# Autodesk Inventor assembly: segment1
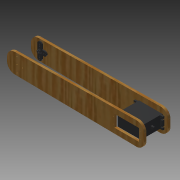
[picture p0: Inventor's stored thumbnail of the model, 180x180]
Saved by Autodesk Inventor 2013 (Build 170138000, 138)
## iProperties
Created: 2014-10-10
Part Number: segment1
Document SubType Name: Assembly
Designer: Masta
Author: Masta
## Documents named in this file (4)
- D:\DrOctopus\3D model\segment1.iam
- D:\DrOctopus\3D model\segment1a.ipt
- D:\DrOctopus\3D model\servo 33kg TGY-S8166M.ipt
- D:\DrOctopus\3D model\servo arm BMS-630MG tripple.ipt
## Components (4 placed, 3 different names)
1. segment1a:1 — Insert:3, Flush:1
2. segment1a:2 — Insert:3, Flush:1, Insert:4, Insert:5, Insert:6, Insert:7
3. servo 33kg TGY-S8166M:1 — Insert:6, Insert:7
4. servo arm BMS-630MG tripple:1 — Insert:4, Insert:5
## Relationships (6: Insert 5, Flush 1)
- Insert:3 (56 mm): segment1a:1 ↔ segment1a:2
- Flush:1: segment1a:1 ↔ segment1a:2
- Insert:4: segment1a:2 ↔ servo arm BMS-630MG tripple:1
- Insert:5: segment1a:2 ↔ servo arm BMS-630MG tripple:1
- Insert:6 (2 mm): segment1a:2 ↔ servo 33kg TGY-S8166M:1
- Insert:7 (2 mm): segment1a:2 ↔ servo 33kg TGY-S8166M:1
